# Autodesk Inventor assembly: IndexerWheelV2
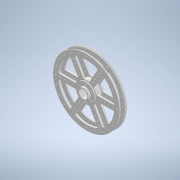
[picture p0: Inventor's stored thumbnail of the model, 180x180]
Saved by Autodesk Inventor 2020 (Build 240168000, 168)
## iProperties
Created: 2020-01-26
Part Number: IndexerWheelV2
Document SubType Name: Assembly
Designer: srini
Author: srini
## Documents named in this file (4)
- C:\Users\srini\Documents\FRC\2020\IntakeShooter\IndexerWheelV2.iam
- C:\Users\srini\Documents\FRC\2020\IntakeShooter\IndexerWheelBushing.ipt
- C:\Users\srini\Documents\FRC\2020\IntakeShooter\IndexerWheelSpacer.ipt
- C:\Users\srini\Documents\FRC\2020\IntakeShooter\IndexerWheelV2.ipt
## Components (5 placed, 3 different names)
1. IndexerWheelBushing:1 — Insert:5
2. IndexerWheelSpacer:1 — Insert:1, Insert:2, Insert:3, Insert:4, Insert:6
3. IndexerWheelV2:1 — Insert:1, Insert:2, Insert:7, Insert:8
4. IndexerWheelV2:2 — Insert:3, Insert:4, Insert:5, Insert:6
5. IndexerWheelBushing:2 — Insert:7, Insert:8
## Relationships (8: Insert 8)
- Insert:1: IndexerWheelSpacer:1 ↔ IndexerWheelV2:1
- Insert:2: IndexerWheelSpacer:1 ↔ IndexerWheelV2:1
- Insert:3: IndexerWheelSpacer:1 ↔ IndexerWheelV2:2
- Insert:4: IndexerWheelSpacer:1 ↔ IndexerWheelV2:2
- Insert:5: IndexerWheelBushing:1 ↔ IndexerWheelV2:2
- Insert:6: IndexerWheelSpacer:1 ↔ IndexerWheelV2:2
- Insert:7: IndexerWheelV2:1 ↔ IndexerWheelBushing:2
- Insert:8: IndexerWheelV2:1 ↔ IndexerWheelBushing:2
